# Autodesk Inventor assembly: Facade12
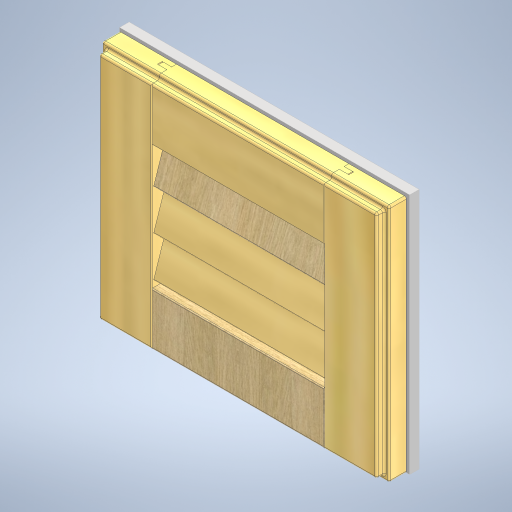
[picture p0: Inventor's stored thumbnail of the model, 512x512]
Saved by Autodesk Inventor 2024 (Build 280153000, 153)
## iProperties
RuleStatus: InUse
AfterAnyParamChange0: FacadeOffsetRule
AfterComponentReplace0: FacadePositionRule
Created: 2019-09-26
Part Number: Facade12
Document SubType Name: Assembly
Designer: RokasM
Author: RokasM
## Documents named in this file (7)
- C:\W4INV 2024 Design\iBOX LIBRARY\Facades\Solid Wood Facade 12\Facade12.iam
- C:\W4INV 2024 Design\iBOX LIBRARY\Facades\Solid Wood Facade 12\box.ipt
- C:\W4INV 2024 Design\iBOX LIBRARY\Facades\Solid Wood Facade 12\blinds.ipt
- C:\W4INV 2024 Design\iBOX LIBRARY\Facades\Solid Wood Facade 12\profile_left.ipt
- C:\W4INV 2024 Design\iBOX LIBRARY\Facades\Solid Wood Facade 12\profile_right.ipt
- C:\W4INV 2024 Design\iBOX LIBRARY\Facades\Solid Wood Facade 12\profile_top.ipt
- C:\W4INV 2024 Design\iBOX LIBRARY\Facades\Solid Wood Facade 12\Facade12.ipt
## Components (9 placed, 6 different names)
1. @Facade12
2. box:1
3. profile_left:1 — Mate:1
4. profile_right:1 — Mate:2, Flush:1
5. profile_top:1
6. profile_top:2 — Mate:1, Mate:2, Flush:1
7. blinds:1
8. blinds:2
9. blinds:3
## Component patterns: blinds_pattern:1 (3 elements)
## Relationships (3: Mate 2, Flush 1)
- Mate:1: profile_left:1 ↔ profile_top:2
- Mate:2: profile_right:1 ↔ profile_top:2
- Flush:1: profile_right:1 ↔ profile_top:2
## Named parameters: cabinet_space_width = 303 mm, cabinet_space_height = 253 mm, top_offset = 0 mm, right_offset = 0 mm, bottom_offset = 0 mm, left_offset = 0 mm, facade_offset = 2 mm, blind_profile_width = 40 mm, blind_profile_thickness = 10 mm, top_tolerance = 1.5 mm, right_tolerance = 1.5 mm, bottom_tolerance = 1.5 mm, left_tolerance = 1.5 mm, blinds = 3, blinds_spacing = 42.33333 mm
